# Autodesk Inventor assembly: ShooterAssemblyWithDartActuator
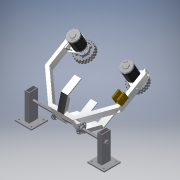
[picture p0: Inventor's stored thumbnail of the model, 180x180]
Saved by Autodesk Inventor 2017 SP1 (Build 210196100, 196)
## iProperties
Created: 2016-02-07
Part Number: ShooterAssemblyWithDartActuator
Document SubType Name: Assembly
Designer: steele
Author: steele
## Documents named in this file (15)
- D:\snobotics\CAD-Development\robSteele\SnoBotics2016\2016-08-05-TiltWithVex\ShooterAssemblyWithDartActuator.iam
- D:\snobotics\CAD-Development\robSteele\SnoBotics2016\2016-05-05-ShooterPrototype\Mini_CIM_MotorHub_4_inch_wheel.iam
- D:\snobotics\CAD-Development\robSteele\SnoBotics2016\2016-05-05-ShooterPrototype\CIM_MotorHub_4_inch_wheel.iam
- D:\snobotics\CAD-Development\robSteele\SnoBotics2016\2016-05-05-ShooterPrototype\ShooterFrameAssembly05.iam
- D:\snobotics\CAD-Development\robSteele\SnoBotics2016\2016-05-05-ShooterPrototype\ShooterAssemblyForRobotV16\Design Accelerator\Bolted Connection1.iam
- D:\snobotics\CAD-Development\robSteele\SnoBotics2016\2016-05-05-ShooterPrototype\ShooterAssemblyForRobotV16\Design Accelerator\Bolted Connection2.iam
- D:\snobotics\CAD-MfgResources\VexRobotics\ThunderHex\217-4002-Hex_1_2x18inch.ipt
- D:\snobotics\CAD-MfgResources\VexRobotics\ThunderHex\217-2592-VersaHub_1_2_inch.ipt
- D:\snobotics\CAD-Development\robSteele\SnoBotics2016\2016-08-05-TiltWithVex\ThunderhexPostWithBearing.iam
- D:\snobotics\CAD-MfgResources\VexRobotics\ThunderHex\217-2737.20121205.ipt
- D:\snobotics\CAD-Development\robSteele\SnoBotics2016\2016-05-05-ShooterPrototype\ShooterAssemblyForRobotV16\Design Accelerator\Bolted Connection6.iam
- D:\snobotics\CAD-Development\robSteele\SnoBotics2016\2016-05-05-ShooterPrototype\ShooterAssemblyForRobotV16\Design Accelerator\Bolted Connection7.iam
- D:\snobotics\CAD-Development\robSteele\SnoBotics2016\2016-05-05-ShooterPrototype\ShooterAssemblyForRobotV16\Design Accelerator\Bolted Connection9.iam
- D:\snobotics\CAD-Development\robSteele\SnoBotics2016\2016-05-05-ShooterPrototype\ShooterAssemblyForRobotV16\Design Accelerator\Bolted Connection10.iam
- D:\snobotics\CAD-Development\robSteele\SnoBotics2016\2016-05-05-ShooterPrototype\BracketForEndOfArm.ipt
## Components (17 placed, 9 different names)
1. ShooterFrameAssembly05:1 [sub-assembly] — Mate:1, Mate:16, Flush:6, Mate:17, Mate:18, Mate:19, Insert:1, Insert:7, Insert:8, Insert:14, Insert:15, Mate:44, Flush:9, Flush:10
2. Mini_CIM_MotorHub_4_inch_wheel:1 [sub-assembly] — Mate:1, Flush:5, Mate:16, Flush:6, Flush:7, Flush:8, Mate:20, Mate:21
3. 217-4002-Hex_1_2x18inch:1 — Insert:1, Insert:3, Insert:4, Insert:5, Insert:6
4. CIM_MotorHub_4_inch_wheel:1 [sub-assembly] — Flush:5, Mate:17, Flush:7, Flush:8
5. Bolted Connection:1 [sub-assembly] — Mate:18, Mate:19
6. Bolted Connection:2 [sub-assembly] — Mate:20, Mate:21
7. 217-2592-VersaHub_1_2_inch:1 — Insert:7, Insert:8, Mate:36, Mate:37, Mate:38, Mate:39
8. 217-2592-VersaHub_1_2_inch:2 — Insert:14, Insert:15, Mate:40, Mate:41, Mate:42, Mate:43
9. ThunderhexPostWithBearing:1 [sub-assembly] — Insert:3
10. ThunderhexPostWithBearing:2 [sub-assembly] — Insert:5
11. 217-2737.20121205:1 — Insert:4
12. 217-2737.20121205:2 — Insert:6
13. Bolted Connection:5 [sub-assembly] — Mate:36, Mate:37
14. Bolted Connection:6 [sub-assembly] — Mate:38, Mate:39
15. Bolted Connection:8 [sub-assembly] — Mate:40, Mate:41
16. Bolted Connection:9 [sub-assembly] — Mate:42, Mate:43
17. BracketForEndOfArm:1 — Mate:44, Flush:9, Flush:10
## Relationships (31: Mate 16, Insert 9, Flush 6)
- Mate:1: ShooterFrameAssembly05:1 ↔ Mini_CIM_MotorHub_4_inch_wheel:1
- Flush:5: Mini_CIM_MotorHub_4_inch_wheel:1 ↔ CIM_MotorHub_4_inch_wheel:1
- Mate:16: ShooterFrameAssembly05:1 ↔ Mini_CIM_MotorHub_4_inch_wheel:1
- Flush:6 (-4.7625 mm): ShooterFrameAssembly05:1 ↔ Mini_CIM_MotorHub_4_inch_wheel:1
- Mate:17: ShooterFrameAssembly05:1 ↔ CIM_MotorHub_4_inch_wheel:1
- Flush:7: Mini_CIM_MotorHub_4_inch_wheel:1 ↔ CIM_MotorHub_4_inch_wheel:1
- Flush:8: Mini_CIM_MotorHub_4_inch_wheel:1 ↔ CIM_MotorHub_4_inch_wheel:1
- Mate:18: ShooterFrameAssembly05:1 ↔ Bolted Connection:1
- Mate:19: ShooterFrameAssembly05:1 ↔ Bolted Connection:1
- Mate:20: Mini_CIM_MotorHub_4_inch_wheel:1 ↔ Bolted Connection:2
- Mate:21: Mini_CIM_MotorHub_4_inch_wheel:1 ↔ Bolted Connection:2
- Insert:1 (152.4 mm): ShooterFrameAssembly05:1 ↔ 217-4002-Hex_1_2x18inch:1
- Insert:3 (-6.35 mm): 217-4002-Hex_1_2x18inch:1 ↔ ThunderhexPostWithBearing:1
- Insert:4: 217-4002-Hex_1_2x18inch:1 ↔ 217-2737.20121205:1
- Insert:5 (-6.35 mm): 217-4002-Hex_1_2x18inch:1 ↔ ThunderhexPostWithBearing:2
- Insert:6: 217-4002-Hex_1_2x18inch:1 ↔ 217-2737.20121205:2
- Insert:7: ShooterFrameAssembly05:1 ↔ 217-2592-VersaHub_1_2_inch:1
- Insert:8: ShooterFrameAssembly05:1 ↔ 217-2592-VersaHub_1_2_inch:1
- Mate:36: 217-2592-VersaHub_1_2_inch:1 ↔ Bolted Connection:5
- Mate:37: 217-2592-VersaHub_1_2_inch:1 ↔ Bolted Connection:5
- Mate:38: 217-2592-VersaHub_1_2_inch:1 ↔ Bolted Connection:6
- Mate:39: 217-2592-VersaHub_1_2_inch:1 ↔ Bolted Connection:6
- Insert:14: ShooterFrameAssembly05:1 ↔ 217-2592-VersaHub_1_2_inch:2
- Insert:15: ShooterFrameAssembly05:1 ↔ 217-2592-VersaHub_1_2_inch:2
- Mate:40: 217-2592-VersaHub_1_2_inch:2 ↔ Bolted Connection:8
- Mate:41: 217-2592-VersaHub_1_2_inch:2 ↔ Bolted Connection:8
- Mate:42: 217-2592-VersaHub_1_2_inch:2 ↔ Bolted Connection:9
- Mate:43: 217-2592-VersaHub_1_2_inch:2 ↔ Bolted Connection:9
- Mate:44: ShooterFrameAssembly05:1 ↔ BracketForEndOfArm:1
- Flush:9 (9.398 mm): ShooterFrameAssembly05:1 ↔ BracketForEndOfArm:1
- Flush:10 (-152.4 mm): ShooterFrameAssembly05:1 ↔ BracketForEndOfArm:1
